# Autodesk Inventor assembly: Assembly1
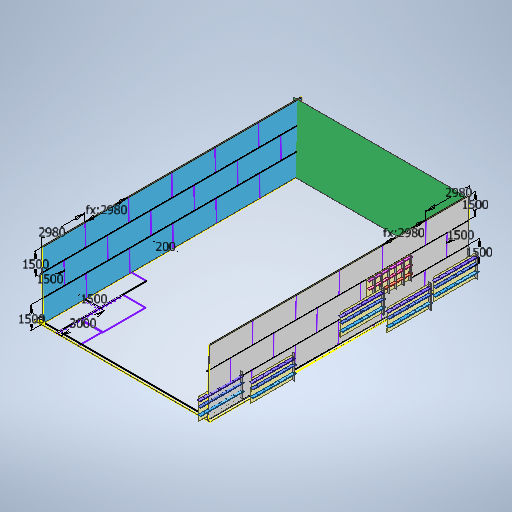
[picture p0: Inventor's stored thumbnail of the model, 512x512]
Saved by Autodesk Inventor 2026.2 (Build 302298000, 298)
## iProperties
Created: 2026-04-17
Part Number: Assembly1
Document SubType Name: Assembly
Designer: admin
Author: admin
## Documents named in this file (6)
- C:\Users\admin\Documents\Inventor\GBK-Gubkinskiy\Assembly1.iam
- C:\Users\admin\Documents\Inventor\GBK-Gubkinskiy\Part1.ipt
- C:\Users\admin\Documents\Inventor\GBK-Gubkinskiy\Assembly shield 1.iam
- C:\Users\admin\Documents\Inventor\GBK-Gubkinskiy\Assembly shield 1_CPY2.iam
- C:\Users\admin\Documents\Inventor\GBK-Gubkinskiy\GBK-Dummy wall1.ipt
- C:\Users\admin\Documents\Inventor\GBK-Gubkinskiy\GBK-Dummy wall 2.ipt
## Components (11 placed, 5 different names)
1. Part1:1 — Mate:9, Mate:10, Mate:11, Mate:12, Mate:13, Mate:14
2. Assembly shield 1:1 [sub-assembly]
3. Assembly shield 1_CPY2:1 [sub-assembly]
4. Assembly shield 1:2 [sub-assembly]
5. Assembly shield 1:3 [sub-assembly]
6. Assembly shield 1:4 [sub-assembly] — Mate:9
7. Assembly shield 1:5 [sub-assembly]
8. Assembly shield 1:6 [sub-assembly]
9. GBK-Dummy wall1:1 — Mate:10
10. GBK-Dummy wall1:2 — Mate:11, Mate:12
11. GBK-Dummy wall 2:1 — Mate:13, Mate:14
## Relationships (8: Mate 7, Flush 1)
- [Flush]: Part1:1 ↔ Assembly shield 1:1
- [Mate]: Part1:1 ↔ Assembly shield 1:1
- Mate:9: Part1:1 ↔ Assembly shield 1:4
- Mate:10: Part1:1 ↔ GBK-Dummy wall1:1
- Mate:11: Part1:1 ↔ GBK-Dummy wall1:2
- Mate:12: Part1:1 ↔ GBK-Dummy wall1:2
- Mate:13: Part1:1 ↔ GBK-Dummy wall 2:1
- Mate:14: Part1:1 ↔ GBK-Dummy wall 2:1
